# Autodesk Inventor assembly: ASY PNS 1720 bottom FDS1 D1200
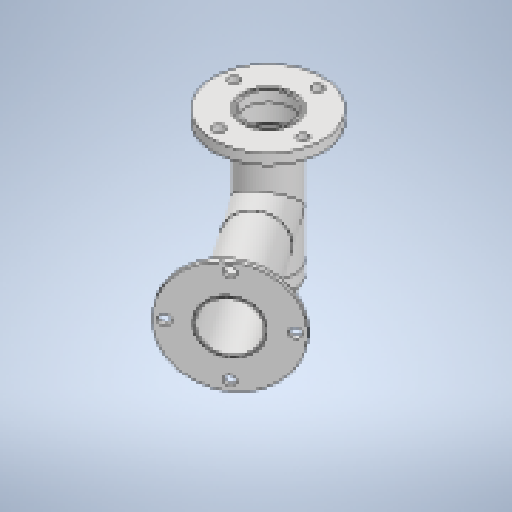
[picture p0: Inventor's stored thumbnail of the model, 512x512]
Saved by Autodesk Inventor 2025.1 (Build 291241020, 241B)
## iProperties
Created: 2025-06-30
Part Number: ASY PNS 1720 bottom FDS1 D1200
Document SubType Name: Assembly
Designer: admin
Author: admin
## Documents named in this file (7)
- C:\Users\user\YandexDisk-badmisterfox\home pc\Inventor\PNS2-Panaevsk\Filter D1200\ASY PNS 1720 bottom FDS1 D1200.iam
- C:\Users\user\YandexDisk-badmisterfox\home pc\Inventor\PNS2-Panaevsk\Filter D1000\DIN 2576 Slip-On Flange for Welding Series 1 (ISO) - PN 10 80 x 88.9.ipt
- C:\Users\user\YandexDisk-badmisterfox\home pc\Inventor\PNS2-Panaevsk\CC\en-US\DIN 2615-1 T\DIN 2615-1 Tee 88.9 x 5.6 S.ipt
- C:\Users\user\YandexDisk-badmisterfox\home pc\Inventor\PNS2-Panaevsk\Filter D1200\PNS 1722 FDS  tube 1.ipt
- C:\Users\user\YandexDisk-badmisterfox\home pc\Inventor\PNS2-Panaevsk\CC\en-US\DIN 2616 CR (K)\DIN 2616 Concentric Reducer (K) 88.9 x 2.3 - 48.3 x 2.ipt
- C:\Users\user\YandexDisk-badmisterfox\home pc\Inventor\PNS2-Panaevsk\Filter D1200\PNS 1723 FDS tube 2.ipt
- C:\Users\user\YandexDisk-badmisterfox\home pc\Inventor\PNS2-Panaevsk\Filter D1200\PNS 1721 FDS flange DN90.ipt
## Components (6 placed, 6 different names)
1. DIN 2576 Slip-On Flange for Welding Series 1 (ISO) - PN 10 80 x 88.9.ipt:1
2. DIN 2615-1 Tee 88.9 x 5.6 S.ipt:1
3. PNS 1722 FDS  tube 1.ipt:1
4. DIN 2616 Concentric Reducer (K) 88.9 x 2.3 - 48.3 x 2.ipt:1
5. PNS 1723 FDS tube 2.ipt:1
6. PNS 1721 FDS flange DN90.ipt:1
## Relationships (5: WeldJoint 4, RevoluteJoint 1)
- [RevoluteJoint]: DIN 2615-1 Tee 88.9 x 5.6 S.ipt:1 ↔ PNS 1722 FDS  tube 1.ipt:1
- [WeldJoint]: DIN 2576 Slip-On Flange for Welding Series 1 (ISO) - PN 10 80 x 88.9.ipt:1 ↔ PNS 1722 FDS  tube 1.ipt:1
- [WeldJoint]: DIN 2615-1 Tee 88.9 x 5.6 S.ipt:1 ↔ DIN 2616 Concentric Reducer (K) 88.9 x 2.3 - 48.3 x 2.ipt:1
- [WeldJoint]: DIN 2615-1 Tee 88.9 x 5.6 S.ipt:1 ↔ PNS 1723 FDS tube 2.ipt:1
- [WeldJoint]: PNS 1723 FDS tube 2.ipt:1 ↔ PNS 1721 FDS flange DN90.ipt:1
